# Autodesk Inventor assembly: Gripper V 10.0 assembly with servo
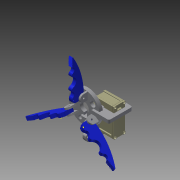
[picture p0: Inventor's stored thumbnail of the model, 180x180]
Saved by Autodesk Inventor 2015 (Build 190159000, 159)
## iProperties
Created: 2015-06-30
Part Number: Gripper V 10.0 assembly with servo
Document SubType Name: Assembly
Designer: Stackpole
Author: Stackpole
## Documents named in this file (9)
- C:\Users\Stackpole\Desktop\Patrick!\Gripper Folder\Gripper V 10.0\Gripper V 10.0 assembly with servo.iam
- C:\Users\Stackpole\Desktop\Patrick!\Gripper Folder\Gripper V 10.0\Gripper V 10.0 base 6mm.ipt
- C:\Users\Stackpole\Desktop\Patrick!\Gripper Folder\Gripper V 10.0\Gripper V 10.0 servo bracket right 6mm.ipt
- C:\Users\Stackpole\Desktop\Patrick!\Gripper Folder\Gripper V 10.0\Gripper V 10.1 servo bracket bottom 6mm.ipt
- C:\Users\Stackpole\Desktop\Patrick!\Gripper Folder\Gripper V 10.0\Gripper V 10.0 servo bracket side left 3mm.ipt
- C:\Users\Stackpole\Desktop\Patrick!\Gripper Folder\Gripper V 10.0\Gripper V 10.0 servo triangle bracket 3mm.ipt
- C:\Users\Stackpole\Desktop\Patrick!\Gripper Folder\Waterproof Servo Assembly.iam
- C:\Users\Stackpole\Desktop\Patrick!\Gripper Folder\Gripper V 10.0\Gripper V 10.0 base tab 3mm.ipt
- C:\Users\Stackpole\Desktop\Patrick!\Gripper Folder\Gripper V 10.0\Gripper V 10.0 finger master 6mm.ipt
## Components (15 placed, 8 different names)
1. Gripper V 10.0 base 6mm:1 — Mate:1, Mate:2, Mate:3, Mate:4, Mate:5, Mate:6, Mate:7, Mate:8, Mate:9, Mate:34, Mate:39, Mate:36, Mate:35, Mate:37, Mate:38, Mate:40, Mate:41, Mate:42, Mate:43, Mate:44, Mate:45, Mate:46, Mate:47, Mate:48, Mate:49, Mate:50, Mate:51
2. Gripper V 10.0 servo bracket right 6mm:1 — Mate:1, Mate:2, Mate:3, Mate:11, Mate:33
3. Gripper V 10.1 servo bracket bottom 6mm:1 — Mate:4, Mate:5, Mate:6, Mate:10, Mate:12, Mate:32
4. Gripper V 10.0 servo bracket side left 3mm:1 — Mate:7, Mate:8, Mate:9
5. Gripper V 10.0 servo triangle bracket 3mm:1 — Mate:10, Mate:11, Mate:12
6. Waterproof Servo Assembly:1 [sub-assembly] — Mate:32, Mate:33, Mate:52
7. Gripper V 10.0 base tab 3mm:1 — Mate:35, Mate:49, Mate:51
8. Gripper V 10.0 base tab 3mm:2 — Mate:36, Mate:41, Mate:42
9. Gripper V 10.0 base tab 3mm:3 — Mate:39, Mate:40, Mate:43, Insert:3
10. Gripper V 10.0 base tab 3mm:4 — Mate:37, Mate:48, Mate:50, Insert:2
11. Gripper V 10.0 base tab 3mm:5 — Mate:38, Mate:45, Mate:46, Insert:1
12. Gripper V 10.0 base tab 3mm:6 — Mate:34, Mate:44, Mate:47
13. Gripper V 10.0 finger master 6mm:1 — Insert:1
14. Gripper V 10.0 finger master 6mm:2 — Insert:2
15. Gripper V 10.0 finger master 6mm:3 — Insert:3
## Relationships (36: Mate 33, Insert 3)
- Mate:1: Gripper V 10.0 base 6mm:1 ↔ Gripper V 10.0 servo bracket right 6mm:1
- Mate:2: Gripper V 10.0 base 6mm:1 ↔ Gripper V 10.0 servo bracket right 6mm:1
- Mate:3: Gripper V 10.0 base 6mm:1 ↔ Gripper V 10.0 servo bracket right 6mm:1
- Mate:4: Gripper V 10.0 base 6mm:1 ↔ Gripper V 10.1 servo bracket bottom 6mm:1
- Mate:5: Gripper V 10.0 base 6mm:1 ↔ Gripper V 10.1 servo bracket bottom 6mm:1
- Mate:6: Gripper V 10.0 base 6mm:1 ↔ Gripper V 10.1 servo bracket bottom 6mm:1
- Mate:7: Gripper V 10.0 base 6mm:1 ↔ Gripper V 10.0 servo bracket side left 3mm:1
- Mate:8: Gripper V 10.0 base 6mm:1 ↔ Gripper V 10.0 servo bracket side left 3mm:1
- Mate:9: Gripper V 10.0 base 6mm:1 ↔ Gripper V 10.0 servo bracket side left 3mm:1
- Mate:10: Gripper V 10.1 servo bracket bottom 6mm:1 ↔ Gripper V 10.0 servo triangle bracket 3mm:1
- Mate:11: Gripper V 10.0 servo bracket right 6mm:1 ↔ Gripper V 10.0 servo triangle bracket 3mm:1
- Mate:12: Gripper V 10.1 servo bracket bottom 6mm:1 ↔ Gripper V 10.0 servo triangle bracket 3mm:1
- Mate:32: Gripper V 10.1 servo bracket bottom 6mm:1 ↔ Waterproof Servo Assembly:1
- Mate:33: Gripper V 10.0 servo bracket right 6mm:1 ↔ Waterproof Servo Assembly:1
- Mate:34: Gripper V 10.0 base 6mm:1 ↔ Gripper V 10.0 base tab 3mm:6
- Mate:39: Gripper V 10.0 base 6mm:1 ↔ Gripper V 10.0 base tab 3mm:3
- Mate:36: Gripper V 10.0 base 6mm:1 ↔ Gripper V 10.0 base tab 3mm:2
- Mate:35: Gripper V 10.0 base 6mm:1 ↔ Gripper V 10.0 base tab 3mm:1
- Mate:37: Gripper V 10.0 base 6mm:1 ↔ Gripper V 10.0 base tab 3mm:4
- Mate:38: Gripper V 10.0 base 6mm:1 ↔ Gripper V 10.0 base tab 3mm:5
- Mate:40: Gripper V 10.0 base 6mm:1 ↔ Gripper V 10.0 base tab 3mm:3
- Mate:41: Gripper V 10.0 base 6mm:1 ↔ Gripper V 10.0 base tab 3mm:2
- Mate:42: Gripper V 10.0 base 6mm:1 ↔ Gripper V 10.0 base tab 3mm:2
- Mate:43: Gripper V 10.0 base 6mm:1 ↔ Gripper V 10.0 base tab 3mm:3
- Mate:44: Gripper V 10.0 base 6mm:1 ↔ Gripper V 10.0 base tab 3mm:6
- Mate:45: Gripper V 10.0 base 6mm:1 ↔ Gripper V 10.0 base tab 3mm:5
- Mate:46: Gripper V 10.0 base 6mm:1 ↔ Gripper V 10.0 base tab 3mm:5
- Mate:47: Gripper V 10.0 base 6mm:1 ↔ Gripper V 10.0 base tab 3mm:6
- Mate:48: Gripper V 10.0 base 6mm:1 ↔ Gripper V 10.0 base tab 3mm:4
- Mate:49: Gripper V 10.0 base 6mm:1 ↔ Gripper V 10.0 base tab 3mm:1
- Mate:50: Gripper V 10.0 base 6mm:1 ↔ Gripper V 10.0 base tab 3mm:4
- Mate:51: Gripper V 10.0 base 6mm:1 ↔ Gripper V 10.0 base tab 3mm:1
- Insert:1: Gripper V 10.0 base tab 3mm:5 ↔ Gripper V 10.0 finger master 6mm:1
- Insert:2: Gripper V 10.0 base tab 3mm:4 ↔ Gripper V 10.0 finger master 6mm:2
- Insert:3: Gripper V 10.0 base tab 3mm:3 ↔ Gripper V 10.0 finger master 6mm:3
- Mate:52 (1370.052 mm): Waterproof Servo Assembly:1
